# Autodesk Inventor assembly: BackAxlePlusWheels
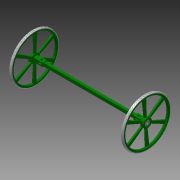
[picture p0: Inventor's stored thumbnail of the model, 180x180]
Saved by Autodesk Inventor 2014 SP1 (Build 180222100, 222)
## iProperties
Created: 2017-01-04
Part Number: BackAxlePlusWheels
Document SubType Name: Assembly
Designer: danielsikar
Author: danielsikar
## Documents named in this file (4)
- C:\Users\danielsikar\Documents\Inventor\IoT-Trike\Assemblies\BackAxlePlusWheels.iam
- C:\Users\danielsikar\Documents\Inventor\IoT-Trike\Assemblies\BackAxleNuts.iam
- C:\Users\danielsikar\Documents\Inventor\IoT-Trike\Assemblies\WheelTyre624Bearing.iam
- C:\Users\danielsikar\Documents\Inventor\IoT-Trike\Assemblies\WheelTyre624Bearing_MIR1.iam
## Components (3 placed, 3 different names)
1. BackAxleNuts:1 [sub-assembly] — Mate:1, Mate:2, Mate:3, Mate:4, Mate:5, Mate:6, Mate:7, Mate:8
2. WheelTyre624Bearing:1 [sub-assembly] — Mate:4, Mate:5
3. WheelTyre624Bearing_MIR1:1 [sub-assembly] — Mate:6, Mate:7
## Relationships (11: Mate 8, Flush 3)
- Mate:1: BackAxleNuts:1
- Mate:2: BackAxleNuts:1
- Mate:3: BackAxleNuts:1
- Mate:4: BackAxleNuts:1 ↔ WheelTyre624Bearing:1
- Mate:5: BackAxleNuts:1 ↔ WheelTyre624Bearing:1
- Flush:1 (137.5 mm)
- Mate:6: BackAxleNuts:1 ↔ WheelTyre624Bearing_MIR1:1
- Mate:7: BackAxleNuts:1 ↔ WheelTyre624Bearing_MIR1:1
- Flush:3 (4 mm)
- Mate:8: BackAxleNuts:1
- Flush:4 (-58.5 mm)
